# Autodesk Inventor assembly: Cryostat
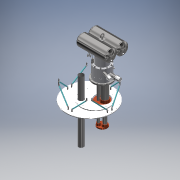
[picture p0: Inventor's stored thumbnail of the model, 180x180]
Saved by Autodesk Inventor 2018 (Build 220112000, 112)
## iProperties
Created: 2018-10-10
Part Number: Cryostat
Document SubType Name: Assembly
Designer: Admin
Author: Admin
## Documents named in this file (9)
- C:\Users\freyja\Documents\Cryorefrigerator\CAD\Cryostat.iam
- C:\Users\freyja\Documents\Cryorefrigerator\CAD\External Models\CH40415 24JUL14 C.ipt
- C:\Users\freyja\Documents\Cryorefrigerator\CAD\vacuum jacket long.ipt
- C:\Users\freyja\Documents\Cryorefrigerator\CAD\vacuum jacket.ipt
- C:\Users\freyja\Documents\Cryorefrigerator\CAD\Top Plate V2.2.ipt
- C:\Users\freyja\Documents\Cryorefrigerator\CAD\still pipe standin.ipt
- C:\Users\freyja\Documents\Cryorefrigerator\CAD\55K stage.ipt
- C:\Users\freyja\Documents\Cryorefrigerator\CAD\mini 55K stage.ipt
- C:\Users\freyja\Documents\Cryorefrigerator\CAD\foot type 3.iam
## Components (15 placed, 8 different names)
1. Top Plate V2.2:1 — Mate:16, Mate:18, Mate:19, Mate:20, Mate:21, Mate:26, Mate:47, Mate:54, Mate:55, Mate:56, Mate:57, Mate:58, Mate:59, Mate:60, Mate:61, Mate:62, Mate:63, Mate:64, Mate:65, Mate:66, Mate:67, Mate:68, Mate:69
2. CH40415 24JUL14 C:1 — Mate:16, Mate:18, Mate:26, Mate:49
3. vacuum jacket long:1 — Mate:7, Mate:8, Mate:9
4. vacuum jacket:1 — Mate:7, Mate:8, Mate:9, Mate:19, Mate:20, Mate:21
5. still pipe standin:1 — Mate:47, Mate:48
6. 55K stage:1 — Mate:51, Mate:52, Mate:53, Mate:70
7. mini 55K stage:1 — Mate:48, Mate:49, Mate:51, Mate:52, Mate:53
8. foot type 3:1 [sub-assembly] — Mate:58, Mate:64
9. foot type 3:2 [sub-assembly] — Mate:56, Mate:68
10. foot type 3:3 [sub-assembly] — Mate:54, Mate:69, Mate:70
11. foot type 3:4 [sub-assembly] — Mate:55, Mate:67
12. foot type 3:5 [sub-assembly] — Mate:57, Mate:66
13. foot type 3:6 [sub-assembly] — Mate:59, Mate:63
14. foot type 3:7 [sub-assembly] — Mate:61, Mate:62
15. foot type 3:8 [sub-assembly] — Mate:60, Mate:65
## Relationships (32: Mate 32)
- Mate:7: vacuum jacket long:1 ↔ vacuum jacket:1
- Mate:8: vacuum jacket long:1 ↔ vacuum jacket:1
- Mate:9: vacuum jacket long:1 ↔ vacuum jacket:1
- Mate:16: Top Plate V2.2:1 ↔ CH40415 24JUL14 C:1
- Mate:18: Top Plate V2.2:1 ↔ CH40415 24JUL14 C:1
- Mate:19: Top Plate V2.2:1 ↔ vacuum jacket:1
- Mate:20: Top Plate V2.2:1 ↔ vacuum jacket:1
- Mate:21: Top Plate V2.2:1 ↔ vacuum jacket:1
- Mate:26: Top Plate V2.2:1 ↔ CH40415 24JUL14 C:1
- Mate:47: Top Plate V2.2:1 ↔ still pipe standin:1
- Mate:48: still pipe standin:1 ↔ mini 55K stage:1
- Mate:49: CH40415 24JUL14 C:1 ↔ mini 55K stage:1
- Mate:51: 55K stage:1 ↔ mini 55K stage:1
- Mate:52: 55K stage:1 ↔ mini 55K stage:1
- Mate:53: 55K stage:1 ↔ mini 55K stage:1
- Mate:54: Top Plate V2.2:1 ↔ foot type 3:3
- Mate:55: Top Plate V2.2:1 ↔ foot type 3:4
- Mate:56: Top Plate V2.2:1 ↔ foot type 3:2
- Mate:57: Top Plate V2.2:1 ↔ foot type 3:5
- Mate:58: Top Plate V2.2:1 ↔ foot type 3:1
- Mate:59: Top Plate V2.2:1 ↔ foot type 3:6
- Mate:60: Top Plate V2.2:1 ↔ foot type 3:8
- Mate:61: Top Plate V2.2:1 ↔ foot type 3:7
- Mate:62: Top Plate V2.2:1 ↔ foot type 3:7
- Mate:63: Top Plate V2.2:1 ↔ foot type 3:6
- Mate:64: Top Plate V2.2:1 ↔ foot type 3:1
- Mate:65: Top Plate V2.2:1 ↔ foot type 3:8
- Mate:66: Top Plate V2.2:1 ↔ foot type 3:5
- Mate:67: Top Plate V2.2:1 ↔ foot type 3:4
- Mate:68: Top Plate V2.2:1 ↔ foot type 3:2
- Mate:69: Top Plate V2.2:1 ↔ foot type 3:3
- Mate:70: 55K stage:1 ↔ foot type 3:3
